# Autodesk Inventor assembly: EDM Machine+Shields
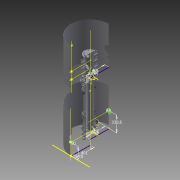
[picture p0: Inventor's stored thumbnail of the model, 180x180]
Saved by Autodesk Inventor 2015 (Build 190159000, 159)
## iProperties
Created: 2014-06-20
Part Number: EDM Machine+Shields
Document SubType Name: Assembly
Designer: Aki
Author: Aki
## Documents named in this file (16)
- C:\ColdMatter\CADFiles\EDM Machine\EDM Machine+Shields.iam
- C:\ColdMatter\CADFiles\EDM Machine\EDM Beamline\Chamber parts\hudson chamber actual size.ipt
- C:\ColdMatter\CADFiles\EDM Machine\EDM Inner Shield\Inner Shield.iam
- C:\ColdMatter\CADFiles\EDM Machine\EDM Beamline\Chamber parts\Centre nipple.iam
- C:\ColdMatter\CADFiles\EDM Machine\Electrical Feedthrough Collar\Electrical Feedthrough Collar.iam
- C:\ColdMatter\CADFiles\EDM Machine\Microwave Detection Region\Microwave Detection Region v2.iam
- C:\ColdMatter\CADFiles\EDM Machine\EDM Middle Shield\EDM Middle Shield Part 1.ipt
- C:\ColdMatter\CADFiles\EDM Machine\EDM Middle Shield\EDM Middle Shield Part 2.ipt
- C:\ColdMatter\CADFiles\EDM Machine\EDM Middle Shield\EDM Middle Shield Part 3.ipt
- C:\ColdMatter\CADFiles\EDM Machine\EDM Middle Shield\EDM Middle Shield Part 4.ipt
- C:\ColdMatter\CADFiles\EDM Machine\EDM Outer Shield\Lower Back Half.ipt
- C:\ColdMatter\CADFiles\EDM Machine\EDM Outer Shield\Lower Front Half.ipt
- C:\ColdMatter\CADFiles\EDM Machine\EDM Outer Shield\Upper Back Half.ipt
- C:\ColdMatter\CADFiles\EDM Machine\EDM Outer Shield\Upper Front Half.ipt
- C:\ColdMatter\CADFiles\EDM Machine\EDM Outer Shield\New Band Design.ipt
- C:\ColdMatter\CADFiles\EDM Machine\Microwave Detection Region\Probe Shield\Probe Shield Design.iam
## Components (16 placed, 15 different names)
1. Inner Shield:1 [sub-assembly] — Mate:2, Mate:8, Mate:13, Mate:14
2. Centre nipple:1 [sub-assembly] — Mate:7, Rotational:1, Mate:15
3. Electrical Feedthrough Collar:1 [sub-assembly] — Rotational:1, Mate:10
4. Microwave Detection Region v2:1 [sub-assembly] — Mate:10
5. hudson chamber actual size:1 — Mate:13, Mate:14, Mate:15, Mate:33, Mate:49, Mate:51
6. EDM Middle Shield Part 1:1 — Mate:18, Mate:19, Mate:20, Mate:23, Mate:25, Mate:27, Mate:33, Mate:37, Mate:45
7. EDM Middle Shield Part 2:1 — Mate:18, Mate:19, Mate:21, Mate:22
8. EDM Middle Shield Part 3:1 — Mate:20, Mate:21, Mate:22, Mate:24, Mate:28
9. EDM Middle Shield Part 4:1 — Mate:23, Mate:24, Mate:25
10. Lower Back Half:1 — Mate:28, Mate:50, Mate:51
11. Lower Front Half:1 — Mate:49, Mate:50
12. Upper Back Half:1 — Mate:39, Mate:40, Mate:44, Mate:48
13. Upper Front Half:4 — Mate:37, Mate:39, Mate:40, Mate:42
14. New Band Design:1 — Mate:42, Mate:44
15. New Band Design:2 — Mate:45
16. Probe Shield Design:1 [sub-assembly] — Mate:48
## Relationships (29: Mate 28, RevoluteJoint 1)
- Mate:2: Inner Shield:1
- Mate:7: Centre nipple:1
- Mate:8: Inner Shield:1
- Rotational:1 [RevoluteJoint]: Centre nipple:1 ↔ Electrical Feedthrough Collar:1
- Mate:10: Electrical Feedthrough Collar:1 ↔ Microwave Detection Region v2:1
- Mate:13: Inner Shield:1 ↔ hudson chamber actual size:1
- Mate:14: Inner Shield:1 ↔ hudson chamber actual size:1
- Mate:15: Centre nipple:1 ↔ hudson chamber actual size:1
- Mate:18: EDM Middle Shield Part 1:1 ↔ EDM Middle Shield Part 2:1
- Mate:19: EDM Middle Shield Part 1:1 ↔ EDM Middle Shield Part 2:1
- Mate:20: EDM Middle Shield Part 1:1 ↔ EDM Middle Shield Part 3:1
- Mate:21: EDM Middle Shield Part 2:1 ↔ EDM Middle Shield Part 3:1
- Mate:22: EDM Middle Shield Part 2:1 ↔ EDM Middle Shield Part 3:1
- Mate:23: EDM Middle Shield Part 1:1 ↔ EDM Middle Shield Part 4:1
- Mate:24: EDM Middle Shield Part 3:1 ↔ EDM Middle Shield Part 4:1
- Mate:25: EDM Middle Shield Part 1:1 ↔ EDM Middle Shield Part 4:1
- Mate:27: EDM Middle Shield Part 1:1
- Mate:28: EDM Middle Shield Part 3:1 ↔ Lower Back Half:1
- Mate:33: hudson chamber actual size:1 ↔ EDM Middle Shield Part 1:1
- Mate:37: EDM Middle Shield Part 1:1 ↔ Upper Front Half:4
- Mate:39: Upper Back Half:1 ↔ Upper Front Half:4
- Mate:40: Upper Back Half:1 ↔ Upper Front Half:4
- Mate:42: Upper Front Half:4 ↔ New Band Design:1
- Mate:44: Upper Back Half:1 ↔ New Band Design:1
- Mate:45: EDM Middle Shield Part 1:1 ↔ New Band Design:2
- Mate:48: Upper Back Half:1 ↔ Probe Shield Design:1
- Mate:49: hudson chamber actual size:1 ↔ Lower Front Half:1
- Mate:50: Lower Back Half:1 ↔ Lower Front Half:1
- Mate:51: hudson chamber actual size:1 ↔ Lower Back Half:1
